# Autodesk Inventor assembly: ELEV_000_FULLASMBLY
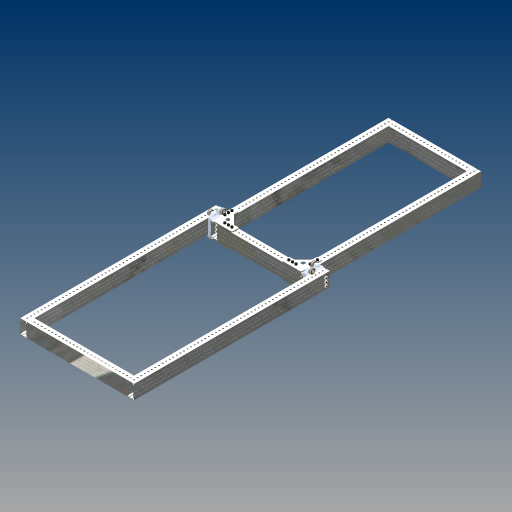
[picture p0: Inventor's stored thumbnail of the model, 512x512]
Saved by Autodesk Inventor 2024.3 (Build 283343000, 343)
## iProperties
Created: 2024-11-25
Part Number: ELEV_000_FULLASMBLY
Document SubType Name: Assembly
Designer: Kenji
Mass: 3407.89 g
Surface Area: 12378 cm^2
Volume: 1206.36 cm^3
Density: 2.82493 g/cm^3
Author: Kenji
## Documents named in this file (18)
- C:\Users\Kenji\Documents\GitHub\1622-2024-Casino-Clash-CAD-A-Thon\Elevator\ELEV_000_FULLASMBLY.iam
- C:\Users\Kenji\Documents\GitHub\1622-2024-Casino-Clash-CAD-A-Thon\Elevator\ELEV_001_BAR1(27.500 in).ipt
- C:\Users\Kenji\Documents\GitHub\1622-2024-Casino-Clash-CAD-A-Thon\Elevator\ELEV_002_BAR2(14.000 in).ipt
- C:\Users\Kenji\Documents\GitHub\1622-2024-Casino-Clash-CAD-A-Thon\Elevator\ELEV_003_BAR3(25.000 in).ipt
- C:\Users\Kenji\Documents\GitHub\1622-2024-Casino-Clash-CAD-A-Thon\COTS Library\Motion\BearingBlocks\ElevatorBlocks\WCP-0897_InlineBearingBlock.iam
- C:\Users\Kenji\Documents\GitHub\1622-2024-Casino-Clash-CAD-A-Thon\Elevator\ELEV_004_BAR4(12.000 in).ipt
- C:\Users\Kenji\Documents\GitHub\1622-2024-Casino-Clash-CAD-A-Thon\Elevator\ELEV_005_SUPBRK1.ipt
- C:\Users\Kenji\Documents\GitHub\1622-2024-Casino-Clash-CAD-A-Thon\COTS Library\Fasteners\Nuts\COTS_90633A411_Low-Strength Steel Thin Nylon-Insert Locknut_10-32.ipt
- C:\Users\Kenji\Documents\GitHub\1622-2024-Casino-Clash-CAD-A-Thon\Elevator\ELEV_006_SUPBRK1_THRD.ipt
- C:\Users\Kenji\Documents\GitHub\1622-2024-Casino-Clash-CAD-A-Thon\COTS Library\Fasteners\Bolts\Socket-Head\10-32\COTS_90044A121_Black-Oxide Alloy Steel Socket Head Screw_10-32_2.5in.ipt
- C:\Users\Kenji\Documents\GitHub\1622-2024-Casino-Clash-CAD-A-Thon\COTS Library\Fasteners\Bolts\Socket-Head\10-32\COTS_90044A202_Black-Oxide Alloy Steel Socket Head Screw_1-.375.ipt
- C:\Users\Kenji\Documents\GitHub\1622-2024-Casino-Clash-CAD-A-Thon\COTS Library\Fasteners\Bolts\Socket-Head\10-32\COTS_91251A342_Black-Oxide Alloy Steel Socket Head Screw_.5in.ipt
- C:\Users\Kenji\Documents\GitHub\1622-2024-Casino-Clash-CAD-A-Thon\Elevator\ELEV_000_FULLASMBLY\AIP\FEA\ew6g7bhkw.fins
- C:\Users\Kenji\Documents\GitHub\1622-2024-Casino-Clash-CAD-A-Thon\Elevator\ELEV_000_FULLASMBLY\AIP\FEA\ew6g7bhkw.fsat
- C:\Users\Kenji\Documents\GitHub\1622-2024-Casino-Clash-CAD-A-Thon\Elevator\ELEV_000_FULLASMBLY\AIP\FEA\ew6g7bhkw.ftes
- C:\Users\Kenji\Documents\GitHub\1622-2024-Casino-Clash-CAD-A-Thon\Elevator\ELEV_000_FULLASMBLY\AIP\FEA\ew6g7bhkw.fwiz
- C:\Users\Kenji\Documents\GitHub\1622-2024-Casino-Clash-CAD-A-Thon\Elevator\ELEV_000_FULLASMBLY\AIP\FEA\ew6g7biao.fmsh
- C:\Users\Kenji\Documents\GitHub\1622-2024-Casino-Clash-CAD-A-Thon\Elevator\ELEV_000_FULLASMBLY\AIP\FEA\ew6g7bibk.fres
## Components (51 placed, 11 different names)
1. ELEV_001_BAR1(27.500 in):1 — Flush:1, Flush:2, Mate:1, Mate:2, Flush:7, Tangent:2, Mate:10, Flush:11, Mate:11, Mate:78
2. ELEV_001_BAR1(27.500 in):2 — Flush:1, Flush:2, Mate:1, Flush:3, Flush:4, Mate:3, Angle:1, Mate:4, Flush:8, Angle:2, Mate:74
3. ELEV_002_BAR2(14.000 in):1 — Flush:3, Flush:4, Mate:2
4. ELEV_003_BAR3(25.000 in):1 — Flush:5, Flush:6, Flush:7, Mate:8, Flush:10, Mate:9, Mate:82
5. ELEV_003_BAR3(25.000 in):2 — Flush:5, Flush:6, Tangent:1, Angle:2, Mate:5, Angle:3, Mate:6, Flush:9, Mate:12, Flush:12, Flush:13, Mate:13, Flush:14, Mate:14, Mate:16, Mate:62, Mate:86
6. WCP-0897_InlineBearingBlock:1 [sub-assembly] — Mate:5, Angle:3, Mate:6, Flush:9, Mate:83, Mate:84
7. WCP-0897_InlineBearingBlock:2 [sub-assembly] — Mate:3, Angle:1, Mate:4, Tangent:1, Flush:8, Mate:71, Mate:72
8. WCP-0897_InlineBearingBlock:3 [sub-assembly] — Mate:8, Flush:10, Mate:9, Tangent:2, Mate:37, Mate:79, Mate:80
9. WCP-0897_InlineBearingBlock:4 [sub-assembly] — Mate:10, Flush:11, Mate:11, Mate:37, Mate:75, Mate:76
10. ELEV_004_BAR4(12.000 in):1 — Mate:12, Flush:12, Flush:13, Mate:17, Mate:18, Mate:19, Angle:4, Mate:20, Mate:42, Mate:45, Mate:60, Flush:15, Mate:61
11. ELEV_004_BAR4(12.000 in):2 — Mate:13, Flush:14, Mate:14
12. ELEV_005_SUPBRK1:1 — Mate:16, Mate:17, Mate:18, Mate:67, Mate:68, Mate:69, Mate:70
13. ELEV_005_SUPBRK1:2 — Mate:19, Angle:4, Mate:20, Mate:63, Mate:64, Mate:65, Mate:66
14. ELEV_006_SUPBRK1_THRD:1 — Mate:42, Mate:61, Mate:62
15. ELEV_006_SUPBRK1_THRD:2 — Mate:45, Mate:60, Flush:15
16. COTS_90044A121_Black-Oxide Alloy Steel Socket Head Screw_10-32_2.5in:1 — Mate:63, Mate:64
17. COTS_90044A121_Black-Oxide Alloy Steel Socket Head Screw_10-32_2.5in:5
18. COTS_90044A121_Black-Oxide Alloy Steel Socket Head Screw_10-32_2.5in:6
19. COTS_90044A121_Black-Oxide Alloy Steel Socket Head Screw_10-32_2.5in:4 — Mate:65, Mate:66
20. COTS_90044A121_Black-Oxide Alloy Steel Socket Head Screw_10-32_2.5in:7
21. COTS_90044A121_Black-Oxide Alloy Steel Socket Head Screw_10-32_2.5in:8
22. COTS_90044A121_Black-Oxide Alloy Steel Socket Head Screw_10-32_2.5in:3 — Mate:68, Mate:70
23. COTS_90044A121_Black-Oxide Alloy Steel Socket Head Screw_10-32_2.5in:9
24. COTS_90044A121_Black-Oxide Alloy Steel Socket Head Screw_10-32_2.5in:10
25. COTS_90044A121_Black-Oxide Alloy Steel Socket Head Screw_10-32_2.5in:2 — Mate:67, Mate:69
26. COTS_90044A121_Black-Oxide Alloy Steel Socket Head Screw_10-32_2.5in:11
27. COTS_90044A121_Black-Oxide Alloy Steel Socket Head Screw_10-32_2.5in:12
28. COTS_90044A202_Black-Oxide Alloy Steel Socket Head Screw_1-.375:1 — Mate:71, Mate:72, Mate:73
29. COTS_90633A411_Low-Strength Steel Thin Nylon-Insert Locknut_10-32:1 — Mate:73, Mate:74
30. COTS_90044A202_Black-Oxide Alloy Steel Socket Head Screw_1-.375:2
31. COTS_90633A411_Low-Strength Steel Thin Nylon-Insert Locknut_10-32:2
32. COTS_90044A202_Black-Oxide Alloy Steel Socket Head Screw_1-.375:3
33. COTS_90633A411_Low-Strength Steel Thin Nylon-Insert Locknut_10-32:3
34. COTS_90633A411_Low-Strength Steel Thin Nylon-Insert Locknut_10-32:4 — Mate:77, Mate:78
35. COTS_90044A202_Black-Oxide Alloy Steel Socket Head Screw_1-.375:4 — Mate:75, Mate:76, Mate:77
36. COTS_90633A411_Low-Strength Steel Thin Nylon-Insert Locknut_10-32:5
37. COTS_90044A202_Black-Oxide Alloy Steel Socket Head Screw_1-.375:5
38. COTS_90633A411_Low-Strength Steel Thin Nylon-Insert Locknut_10-32:6
39. COTS_90044A202_Black-Oxide Alloy Steel Socket Head Screw_1-.375:6
40. COTS_91251A342_Black-Oxide Alloy Steel Socket Head Screw_.5in:1 — Mate:79, Mate:80, Mate:81
41. COTS_90633A411_Low-Strength Steel Thin Nylon-Insert Locknut_10-32:7 — Mate:81, Mate:82
42. COTS_91251A342_Black-Oxide Alloy Steel Socket Head Screw_.5in:2
43. COTS_90633A411_Low-Strength Steel Thin Nylon-Insert Locknut_10-32:8
44. COTS_91251A342_Black-Oxide Alloy Steel Socket Head Screw_.5in:3
45. COTS_90633A411_Low-Strength Steel Thin Nylon-Insert Locknut_10-32:9
46. COTS_90633A411_Low-Strength Steel Thin Nylon-Insert Locknut_10-32:10 — Mate:85, Mate:86
47. COTS_91251A342_Black-Oxide Alloy Steel Socket Head Screw_.5in:4 — Mate:83, Mate:84, Mate:85
48. COTS_90633A411_Low-Strength Steel Thin Nylon-Insert Locknut_10-32:11
49. COTS_91251A342_Black-Oxide Alloy Steel Socket Head Screw_.5in:5
50. COTS_90633A411_Low-Strength Steel Thin Nylon-Insert Locknut_10-32:12
51. COTS_91251A342_Black-Oxide Alloy Steel Socket Head Screw_.5in:6
## Component patterns: (3 elements, first: COTS_90044A121_Black-Oxide Alloy Steel Socket Head Screw_10-32_2.5in:1), (3 elements, first: COTS_90044A121_Black-Oxide Alloy Steel Socket Head Screw_10-32_2.5in:4), (3 elements, first: COTS_90044A121_Black-Oxide Alloy Steel Socket Head Screw_10-32_2.5in:3), (3 elements, first: COTS_90044A121_Black-Oxide Alloy Steel Socket Head Screw_10-32_2.5in:2), (3 elements, first: COTS_90044A202_Black-Oxide Alloy Steel Socket Head Screw_1-.375:1 + COTS_90633A411_Low-Strength Steel Thin Nylon-Insert Locknut_10-32:1), (3 elements, first: COTS_90633A411_Low-Strength Steel Thin Nylon-Insert Locknut_10-32:4 + COTS_90044A202_Black-Oxide Alloy Steel Socket Head Screw_1-.375:4), (3 elements, first: COTS_91251A342_Black-Oxide Alloy Steel Socket Head Screw_.5in:1 + COTS_90633A411_Low-Strength Steel Thin Nylon-Insert Locknut_10-32:7), (3 elements, first: COTS_90633A411_Low-Strength Steel Thin Nylon-Insert Locknut_10-32:10 + COTS_91251A342_Black-Oxide Alloy Steel Socket Head Screw_.5in:4)
## Relationships (69: Mate 48, Flush 15, Angle 4, Tangent 2)
- Flush:1: ELEV_001_BAR1(27.500 in):1 ↔ ELEV_001_BAR1(27.500 in):2
- Flush:2: ELEV_001_BAR1(27.500 in):1 ↔ ELEV_001_BAR1(27.500 in):2
- Mate:1 (355.6 mm): ELEV_001_BAR1(27.500 in):1 ↔ ELEV_001_BAR1(27.500 in):2
- Flush:3: ELEV_001_BAR1(27.500 in):2 ↔ ELEV_002_BAR2(14.000 in):1
- Flush:4: ELEV_001_BAR1(27.500 in):2 ↔ ELEV_002_BAR2(14.000 in):1
- Mate:2: ELEV_001_BAR1(27.500 in):1 ↔ ELEV_002_BAR2(14.000 in):1
- Flush:5: ELEV_003_BAR3(25.000 in):1 ↔ ELEV_003_BAR3(25.000 in):2
- Flush:6: ELEV_003_BAR3(25.000 in):1 ↔ ELEV_003_BAR3(25.000 in):2
- Flush:7: ELEV_001_BAR1(27.500 in):1 ↔ ELEV_003_BAR3(25.000 in):1
- Mate:3: ELEV_001_BAR1(27.500 in):2 ↔ WCP-0897_InlineBearingBlock:2
- Angle:1 (0 deg): ELEV_001_BAR1(27.500 in):2 ↔ WCP-0897_InlineBearingBlock:2
- Mate:4: ELEV_001_BAR1(27.500 in):2 ↔ WCP-0897_InlineBearingBlock:2
- Tangent:1: ELEV_003_BAR3(25.000 in):2 ↔ WCP-0897_InlineBearingBlock:2
- Flush:8: ELEV_001_BAR1(27.500 in):2 ↔ WCP-0897_InlineBearingBlock:2
- Angle:2 (0 deg): ELEV_001_BAR1(27.500 in):2 ↔ ELEV_003_BAR3(25.000 in):2
- Mate:5: ELEV_003_BAR3(25.000 in):2 ↔ WCP-0897_InlineBearingBlock:1
- Angle:3 (0 deg): ELEV_003_BAR3(25.000 in):2 ↔ WCP-0897_InlineBearingBlock:1
- Mate:6: ELEV_003_BAR3(25.000 in):2 ↔ WCP-0897_InlineBearingBlock:1
- Flush:9: ELEV_003_BAR3(25.000 in):2 ↔ WCP-0897_InlineBearingBlock:1
- Mate:8: ELEV_003_BAR3(25.000 in):1 ↔ WCP-0897_InlineBearingBlock:3
- Flush:10: ELEV_003_BAR3(25.000 in):1 ↔ WCP-0897_InlineBearingBlock:3
- Mate:9: ELEV_003_BAR3(25.000 in):1 ↔ WCP-0897_InlineBearingBlock:3
- Tangent:2: ELEV_001_BAR1(27.500 in):1 ↔ WCP-0897_InlineBearingBlock:3
- Mate:10: ELEV_001_BAR1(27.500 in):1 ↔ WCP-0897_InlineBearingBlock:4
- Flush:11: ELEV_001_BAR1(27.500 in):1 ↔ WCP-0897_InlineBearingBlock:4
- Mate:11: ELEV_001_BAR1(27.500 in):1 ↔ WCP-0897_InlineBearingBlock:4
- Mate:12: ELEV_003_BAR3(25.000 in):2 ↔ ELEV_004_BAR4(12.000 in):1
- Flush:12: ELEV_003_BAR3(25.000 in):2 ↔ ELEV_004_BAR4(12.000 in):1
- Flush:13: ELEV_003_BAR3(25.000 in):2 ↔ ELEV_004_BAR4(12.000 in):1
- Mate:13: ELEV_003_BAR3(25.000 in):2 ↔ ELEV_004_BAR4(12.000 in):2
- Flush:14: ELEV_003_BAR3(25.000 in):2 ↔ ELEV_004_BAR4(12.000 in):2
- Mate:14: ELEV_003_BAR3(25.000 in):2 ↔ ELEV_004_BAR4(12.000 in):2
- Mate:16: ELEV_003_BAR3(25.000 in):2 ↔ ELEV_005_SUPBRK1:1
- Mate:17: ELEV_004_BAR4(12.000 in):1 ↔ ELEV_005_SUPBRK1:1
- Mate:18: ELEV_004_BAR4(12.000 in):1 ↔ ELEV_005_SUPBRK1:1
- Mate:19: ELEV_004_BAR4(12.000 in):1 ↔ ELEV_005_SUPBRK1:2
- Angle:4 (0 deg): ELEV_004_BAR4(12.000 in):1 ↔ ELEV_005_SUPBRK1:2
- Mate:20: ELEV_004_BAR4(12.000 in):1 ↔ ELEV_005_SUPBRK1:2
- Mate:37: WCP-0897_InlineBearingBlock:3 ↔ WCP-0897_InlineBearingBlock:4
- Mate:42: ELEV_004_BAR4(12.000 in):1 ↔ ELEV_006_SUPBRK1_THRD:1
- Mate:45: ELEV_004_BAR4(12.000 in):1 ↔ ELEV_006_SUPBRK1_THRD:2
- Mate:60: ELEV_004_BAR4(12.000 in):1 ↔ ELEV_006_SUPBRK1_THRD:2
- Flush:15: ELEV_004_BAR4(12.000 in):1 ↔ ELEV_006_SUPBRK1_THRD:2
- Mate:61: ELEV_004_BAR4(12.000 in):1 ↔ ELEV_006_SUPBRK1_THRD:1
- Mate:62: ELEV_003_BAR3(25.000 in):2 ↔ ELEV_006_SUPBRK1_THRD:1
- Mate:63: ELEV_005_SUPBRK1:2 ↔ COTS_90044A121_Black-Oxide Alloy Steel Socket Head Screw_10-32_2.5in:1
- Mate:64: ELEV_005_SUPBRK1:2 ↔ COTS_90044A121_Black-Oxide Alloy Steel Socket Head Screw_10-32_2.5in:1
- Mate:65: ELEV_005_SUPBRK1:2 ↔ COTS_90044A121_Black-Oxide Alloy Steel Socket Head Screw_10-32_2.5in:4
- Mate:66: ELEV_005_SUPBRK1:2 ↔ COTS_90044A121_Black-Oxide Alloy Steel Socket Head Screw_10-32_2.5in:4
- Mate:67: ELEV_005_SUPBRK1:1 ↔ COTS_90044A121_Black-Oxide Alloy Steel Socket Head Screw_10-32_2.5in:2
- Mate:68: ELEV_005_SUPBRK1:1 ↔ COTS_90044A121_Black-Oxide Alloy Steel Socket Head Screw_10-32_2.5in:3
- Mate:69: ELEV_005_SUPBRK1:1 ↔ COTS_90044A121_Black-Oxide Alloy Steel Socket Head Screw_10-32_2.5in:2
- Mate:70: ELEV_005_SUPBRK1:1 ↔ COTS_90044A121_Black-Oxide Alloy Steel Socket Head Screw_10-32_2.5in:3
- Mate:71: WCP-0897_InlineBearingBlock:2 ↔ COTS_90044A202_Black-Oxide Alloy Steel Socket Head Screw_1-.375:1
- Mate:72: WCP-0897_InlineBearingBlock:2 ↔ COTS_90044A202_Black-Oxide Alloy Steel Socket Head Screw_1-.375:1
- Mate:73: COTS_90044A202_Black-Oxide Alloy Steel Socket Head Screw_1-.375:1 ↔ COTS_90633A411_Low-Strength Steel Thin Nylon-Insert Locknut_10-32:1
- Mate:74: ELEV_001_BAR1(27.500 in):2 ↔ COTS_90633A411_Low-Strength Steel Thin Nylon-Insert Locknut_10-32:1
- Mate:75: WCP-0897_InlineBearingBlock:4 ↔ COTS_90044A202_Black-Oxide Alloy Steel Socket Head Screw_1-.375:4
- Mate:76: WCP-0897_InlineBearingBlock:4 ↔ COTS_90044A202_Black-Oxide Alloy Steel Socket Head Screw_1-.375:4
- Mate:77: COTS_90633A411_Low-Strength Steel Thin Nylon-Insert Locknut_10-32:4 ↔ COTS_90044A202_Black-Oxide Alloy Steel Socket Head Screw_1-.375:4
- Mate:78: ELEV_001_BAR1(27.500 in):1 ↔ COTS_90633A411_Low-Strength Steel Thin Nylon-Insert Locknut_10-32:4
- Mate:79: WCP-0897_InlineBearingBlock:3 ↔ COTS_91251A342_Black-Oxide Alloy Steel Socket Head Screw_.5in:1
- Mate:80: WCP-0897_InlineBearingBlock:3 ↔ COTS_91251A342_Black-Oxide Alloy Steel Socket Head Screw_.5in:1
- Mate:81: COTS_91251A342_Black-Oxide Alloy Steel Socket Head Screw_.5in:1 ↔ COTS_90633A411_Low-Strength Steel Thin Nylon-Insert Locknut_10-32:7
- Mate:82: ELEV_003_BAR3(25.000 in):1 ↔ COTS_90633A411_Low-Strength Steel Thin Nylon-Insert Locknut_10-32:7
- Mate:83: WCP-0897_InlineBearingBlock:1 ↔ COTS_91251A342_Black-Oxide Alloy Steel Socket Head Screw_.5in:4
- Mate:84: WCP-0897_InlineBearingBlock:1 ↔ COTS_91251A342_Black-Oxide Alloy Steel Socket Head Screw_.5in:4
- Mate:85: COTS_90633A411_Low-Strength Steel Thin Nylon-Insert Locknut_10-32:10 ↔ COTS_91251A342_Black-Oxide Alloy Steel Socket Head Screw_.5in:4
- Mate:86: ELEV_003_BAR3(25.000 in):2 ↔ COTS_90633A411_Low-Strength Steel Thin Nylon-Insert Locknut_10-32:10
## Named parameters: sa_0 = 35585.8
note: some values were not read from the file. Shown as the stored number, unit unknown: "sa_0".
